# Autodesk Inventor assembly: Сборка_сервопривода
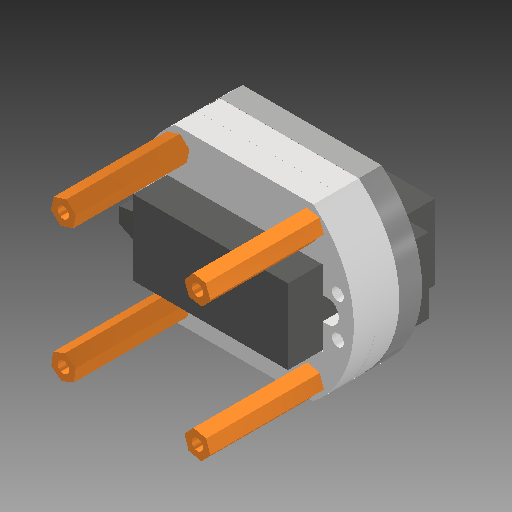
[picture p0: Inventor's stored thumbnail of the model, 512x512]
Saved by Autodesk Inventor 2022 (Build 260153000, 153)
## iProperties
Created: 2025-01-18
Part Number: Сборка_сервопривода
Document SubType Name: Assembly
Designer: Ivan
Mass: 60.2614 g
Surface Area: 264.779 cm^2
Volume: 60.2614 cm^3
Density: 1 g/cm^3
Author: Ivan
Title: Сборка_сервопривода
## Documents named in this file (4)
- E:\Предпроф 2025\Shoter_1_ZIP\Сборка_сервопривода.iam
- E:\Предпроф 2025\Shoter_1_ZIP\Кронштейн_сервопривод.ipt
- E:\Предпроф 2025\Shoter_1_ZIP\1.ipt
- E:\Предпроф 2025\Shoter_1_ZIP\Стойка м3х40.ipt
## Components (8 placed, 3 different names)
1. Кронштейн_сервопривод:1 — Совмещение:4, Заподлицо:1, Совмещение:5, Совмещение:8, Совмещение:9, Совмещение:10, Совмещение:11, Совмещение:12, Совмещение:16, Совмещение:17, Совмещение:18, Совмещение:19
2. 1:1 — Совмещение:6, Совмещение:8, Совмещение:9
3. Кронштейн_сервопривод:2 — Совмещение:10, Совмещение:11, Совмещение:12, Совмещение:13, Совмещение:14, Совмещение:15
4. Кронштейн_сервопривод:3 — Совмещение:13, Совмещение:14, Совмещение:15, Совмещение:20, Совмещение:21, Совмещение:22, Совмещение:23
5. Стойка м3х40:1 — Совмещение:17, Совмещение:21
6. Стойка м3х40:2 — Совмещение:19, Совмещение:22
7. Стойка м3х40:3 — Совмещение:18, Совмещение:23
8. Стойка м3х40:4 — Совмещение:16, Совмещение:20
## Relationships (20: Mate 19, Flush 1)
- Совмещение:4 [Mate]: Кронштейн_сервопривод:1
- Заподлицо:1 [Flush]: Кронштейн_сервопривод:1
- Совмещение:5 [Mate]: Кронштейн_сервопривод:1
- Совмещение:6 [Mate]: 1:1
- Совмещение:8 [Mate] (0.35 mm): Кронштейн_сервопривод:1 ↔ 1:1
- Совмещение:9 [Mate]: Кронштейн_сервопривод:1 ↔ 1:1
- Совмещение:10 [Mate]: Кронштейн_сервопривод:1 ↔ Кронштейн_сервопривод:2
- Совмещение:11 [Mate]: Кронштейн_сервопривод:1 ↔ Кронштейн_сервопривод:2
- Совмещение:12 [Mate]: Кронштейн_сервопривод:1 ↔ Кронштейн_сервопривод:2
- Совмещение:13 [Mate]: Кронштейн_сервопривод:2 ↔ Кронштейн_сервопривод:3
- Совмещение:14 [Mate]: Кронштейн_сервопривод:2 ↔ Кронштейн_сервопривод:3
- Совмещение:15 [Mate]: Кронштейн_сервопривод:2 ↔ Кронштейн_сервопривод:3
- Совмещение:16 [Mate]: Кронштейн_сервопривод:1 ↔ Стойка м3х40:4
- Совмещение:17 [Mate]: Кронштейн_сервопривод:1 ↔ Стойка м3х40:1
- Совмещение:18 [Mate]: Кронштейн_сервопривод:1 ↔ Стойка м3х40:3
- Совмещение:19 [Mate]: Кронштейн_сервопривод:1 ↔ Стойка м3х40:2
- Совмещение:20 [Mate]: Кронштейн_сервопривод:3 ↔ Стойка м3х40:4
- Совмещение:21 [Mate]: Кронштейн_сервопривод:3 ↔ Стойка м3х40:1
- Совмещение:22 [Mate]: Кронштейн_сервопривод:3 ↔ Стойка м3х40:2
- Совмещение:23 [Mate]: Кронштейн_сервопривод:3 ↔ Стойка м3х40:3
